# Autodesk Inventor assembly: Visual Assembly
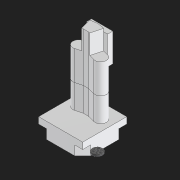
[picture p0: Inventor's stored thumbnail of the model, 180x180]
Saved by Autodesk Inventor 2017 SP1 (Build 210196100, 196)
## iProperties
Created: 2018-03-03
Part Number: Visual Assembly
Document SubType Name: Assembly
Designer: Zach
Author: Zach
## Documents named in this file (4)
- C:\Users\Zach\Documents\GitHub\tr1_description\meshes\Visual Assembly\Visual Assembly.iam
- C:\Users\Zach\Documents\GitHub\tr1_description\meshes\Visual Assembly\Base.ipt
- C:\Users\Zach\Documents\GitHub\tr1_description\meshes\Visual Assembly\Body.ipt
- C:\Users\Zach\Documents\GitHub\tr1_description\meshes\Visual Assembly\Wheel.ipt
## Components (3 placed, 3 different names)
1. Base:1 — Mate:1, Mate:2, Mate:3
2. Body:1 — Mate:1, Mate:2, Mate:3
3. Wheel:1
## Relationships (3: Mate 3)
- Mate:1: Base:1 ↔ Body:1
- Mate:2: Base:1 ↔ Body:1
- Mate:3: Base:1 ↔ Body:1
